# Autodesk Inventor assembly: Application_Incubator_Microscope_v2
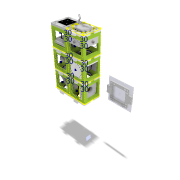
[picture p0: Inventor's stored thumbnail of the model, 180x180]
Saved by Autodesk Inventor 2022 (Build 260153000, 153)
## iProperties
Created: 2019-07-16
Part Number: Application_Incubator_Microscope_v2
Document SubType Name: Assembly
Designer: marsikovabarbora
Author: marsikovabarbora
## Documents named in this file (11)
- C:\Users\diederichbenedict\Dropbox\Dokumente\Promotion\PROJECTS\UC2\02_CAD\INVENTOR\uc2_v3\Application_Incubator_Microscope_v2.iam
- C:\Users\diederichbenedict\Dropbox\Dokumente\Promotion\PROJECTS\UC2\02_CAD\INVENTOR\uc2_v3\Assembly_Cube_Mirror_30x30_v3.iam
- C:\Users\diederichbenedict\Dropbox\Dokumente\Promotion\PROJECTS\UC2\02_CAD\INVENTOR\uc2_v3\Assembly_Cube_RaspiCam_v3.iam
- C:\Users\diederichbenedict\Dropbox\Dokumente\Promotion\PROJECTS\UC2\02_CAD\INVENTOR\uc2_v3\10_Base_puzzle_v3.ipt
- C:\Users\diederichbenedict\Dropbox\Dokumente\Promotion\PROJECTS\UC2\02_CAD\INVENTOR\uc2_v3\Assembly_Cube_LED_Matrix_8x8_v3.iam
- C:\Users\diederichbenedict\Dropbox\Dokumente\Promotion\PROJECTS\UC2\02_CAD\INVENTOR\uc2_v3\Assembly_Cube_empty_IM_withBase_v3.iam
- C:\Users\diederichbenedict\Dropbox\Dokumente\Promotion\PROJECTS\UC2\02_CAD\INVENTOR\uc2_v3\Assembly_Cube_LED_Matrix_v3.iam
- C:\Users\diederichbenedict\Dropbox\Dokumente\Promotion\PROJECTS\UC2\02_CAD\INVENTOR\uc2_v3\Assembly_Cube_Z_Focus_MGN_NEMA_captive_v3.iam
- C:\Users\diederichbenedict\Dropbox\Dokumente\Promotion\PROJECTS\UC2\02_CAD\INVENTOR\uc2_v3\Assembly_Cube_empty_IM_v3.iam
- C:\Users\diederichbenedict\Dropbox\Dokumente\Promotion\PROJECTS\UC2\02_CAD\INVENTOR\uc2_v3\00_objectivelens_10x.ipt
- C:\Users\diederichbenedict\Dropbox\Dokumente\Promotion\PROJECTS\UC2\02_CAD\INVENTOR\uc2_v3\20_Cube_insert_Sample_holder_v3.ipt
## Components (15 placed, 10 different names)
1. Assembly_Cube_Mirror_30x30_v3:1 [sub-assembly] — Mate:11
2. Assembly_Cube_RaspiCam_v3:1 [sub-assembly] — Passend:3, Winkel:1, Passend:4, Passend:7
3. 10_Base_puzzle_v3:5 — Flush:2, Flush:3, Flush:6, Insert:3
4. Assembly_Cube_LED_Matrix_8x8_v3:1 [sub-assembly]
5. Assembly_Cube_empty_IM_withBase_v3:1 [sub-assembly] — Flush:6, Insert:2, Insert:4, Angle:2
6. Assembly_Cube_LED_Matrix_v3:1 [sub-assembly] — Insert:2
7. Assembly_Cube_Z_Focus_MGN_NEMA_captive_v3:1 [sub-assembly] — Insert:3, Insert:5, Insert:6
8. Assembly_Cube_empty_IM_v3:1 [sub-assembly] — Insert:4, Angle:2
9. 10_Base_puzzle_v3:6 — Insert:5
10. 00_objectivelens_10x:1 — Insert:6, Insert:7
11. 20_Cube_insert_Sample_holder_v3:1 — Insert:7
12. 10_Base_puzzle_v3:1 — Passend:7, Flush:2
13. 10_Base_puzzle_v3:3 — Flush:3
14. 10_Base_puzzle_v3:2 — Passend:3, Winkel:1, Passend:4
15. 10_Base_puzzle_v3:4 — Passend:1, Fluchtend:1, Passend:2, Mate:11
## Component patterns: (2 elements, first: 10_Base_puzzle_v3:1), (2 elements, first: 10_Base_puzzle_v3:2)
## Relationships (18: Mate 6, Insert 6, Flush 4, Angle 2)
- Passend:1 [Mate]: 10_Base_puzzle_v3:4
- Fluchtend:1 [Flush]: 10_Base_puzzle_v3:4
- Passend:2 [Mate]: 10_Base_puzzle_v3:4
- Passend:3 [Mate]: Assembly_Cube_RaspiCam_v3:1 ↔ 10_Base_puzzle_v3:2
- Winkel:1 [Angle] (0 deg): Assembly_Cube_RaspiCam_v3:1 ↔ 10_Base_puzzle_v3:2
- Passend:4 [Mate]: Assembly_Cube_RaspiCam_v3:1 ↔ 10_Base_puzzle_v3:2
- Passend:7 [Mate]: Assembly_Cube_RaspiCam_v3:1 ↔ 10_Base_puzzle_v3:1
- Mate:11: Assembly_Cube_Mirror_30x30_v3:1 ↔ 10_Base_puzzle_v3:4
- Flush:2: 10_Base_puzzle_v3:5 ↔ 10_Base_puzzle_v3:1
- Flush:3 (-55 mm): 10_Base_puzzle_v3:5 ↔ 10_Base_puzzle_v3:3
- Flush:6: 10_Base_puzzle_v3:5 ↔ Assembly_Cube_empty_IM_withBase_v3:1
- Insert:2: Assembly_Cube_empty_IM_withBase_v3:1 ↔ Assembly_Cube_LED_Matrix_v3:1
- Insert:3: 10_Base_puzzle_v3:5 ↔ Assembly_Cube_Z_Focus_MGN_NEMA_captive_v3:1
- Insert:4: Assembly_Cube_empty_IM_withBase_v3:1 ↔ Assembly_Cube_empty_IM_v3:1
- Angle:2 (0 deg): Assembly_Cube_empty_IM_withBase_v3:1 ↔ Assembly_Cube_empty_IM_v3:1
- Insert:5: Assembly_Cube_Z_Focus_MGN_NEMA_captive_v3:1 ↔ 10_Base_puzzle_v3:6
- Insert:6: Assembly_Cube_Z_Focus_MGN_NEMA_captive_v3:1 ↔ 00_objectivelens_10x:1
- Insert:7 (-10 mm): 00_objectivelens_10x:1 ↔ 20_Cube_insert_Sample_holder_v3:1
